# Autodesk Inventor assembly: Head
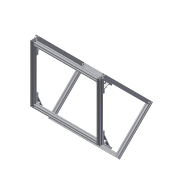
[picture p0: Inventor's stored thumbnail of the model, 180x180]
Saved by Autodesk Inventor 2014 SP1 (Build 180222100, 222)
## iProperties
Created: 2015-02-11
Part Number: Head
Document SubType Name: Assembly
Designer: Simen
Author: Simen
## Documents named in this file (9)
- C:\Users\Simen\Documents\git\Eit\skjellet\Head.iam
- C:\Users\Simen\Documents\git\Eit\skjellet\HBL45TS6hbl45ts6.ipt
- C:\Users\Simen\Documents\git\Eit\skjellet\HBL135TS6.iam
- C:\Users\Simen\Documents\git\Eit\skjellet\KHFS5_2020_386.ipt
- C:\Users\Simen\Documents\git\Eit\skjellet\KHFS5_2020_391.ipt
- C:\Users\Simen\Documents\git\Eit\skjellet\KHFS5_2020_410.ipt
- C:\Users\Simen\Documents\git\Eit\skjellet\HBLFSN5.iam
- C:\Users\Simen\Documents\git\Eit\skjellet\KHFS5_2020_330.ipt
- C:\Users\Simen\Documents\git\Eit\skjellet\KHFS5_2020_101.ipt
## Components (17 placed, 4 different names)
1. HBL45TS6hbl45ts6:1 — Mate:42, Flush:38, Mate:43, Mate:53, Mate:54
2. HBL135TS6:1 [sub-assembly] — Mate:57, Flush:52, Mate:58, Mate:66
3. HBL45TS6hbl45ts6:2 — Mate:41, Flush:39, Mate:44, Mate:55, Mate:56, Flush:51
4. HBL135TS6:2 [sub-assembly] — Mate:69, Flush:67, Mate:72
5. KHFS5-2020-4000:17 — Mate:63, Flush:59, Flush:60, Mate:65, Flush:64, Flush:65
6. KHFS5-2020-4000:18 — Mate:41, Flush:39, Mate:44
7. KHFS5-2020-4000:19 — Mate:42, Flush:38, Mate:43, Flush:50, Flush:56, Mate:62, Flush:58, Flush:61
8. KHFS5-2020-4000:26 — Flush:62, Mate:64, Flush:63, Flush:68, Mate:70, Flush:69
9. KHFS5-2020-4000:27 — Mate:60, Flush:55, Flush:58
10. KHFS5-2020-4000:28 — Mate:59, Flush:53, Flush:54
11. HBLFSN5:1 [sub-assembly] — Mate:61, Flush:57, Mate:68
12. KHFS5-2020-4000:29 — Mate:53, Mate:54, Flush:50, Mate:57, Flush:52, Mate:58, Mate:59, Flush:53, Flush:54, Mate:63, Flush:59, Flush:60
13. KHFS5-2020-4000:30 — Mate:55, Mate:56, Flush:51, Mate:65, Flush:64, Flush:65, Mate:69, Flush:67
14. KHFS5-2020-4000:31 — Mate:60, Flush:55, Flush:56, Mate:61, Flush:57, Mate:62, Flush:61, Flush:62, Mate:64, Flush:63, Mate:67, Flush:66
15. KHFS5-2020-4000:32 — Mate:66, Mate:67, Flush:66, Mate:68
16. KHFS5-2020-4000:33 — Mate:71, Flush:70, Flush:71, Mate:72
17. KHFS5-2020-4000:34 — Flush:68, Mate:70, Flush:69, Mate:71, Flush:70, Flush:71
## Relationships (48: Mate 24, Flush 24)
- Mate:41: HBL45TS6hbl45ts6:2 ↔ KHFS5-2020-4000:18
- Mate:42: HBL45TS6hbl45ts6:1 ↔ KHFS5-2020-4000:19
- Flush:38: HBL45TS6hbl45ts6:1 ↔ KHFS5-2020-4000:19
- Flush:39: HBL45TS6hbl45ts6:2 ↔ KHFS5-2020-4000:18
- Mate:43: HBL45TS6hbl45ts6:1 ↔ KHFS5-2020-4000:19
- Mate:44: HBL45TS6hbl45ts6:2 ↔ KHFS5-2020-4000:18
- Mate:53: HBL45TS6hbl45ts6:1 ↔ KHFS5-2020-4000:29
- Mate:54: HBL45TS6hbl45ts6:1 ↔ KHFS5-2020-4000:29
- Flush:50: KHFS5-2020-4000:19 ↔ KHFS5-2020-4000:29
- Mate:55: HBL45TS6hbl45ts6:2 ↔ KHFS5-2020-4000:30
- Mate:56: HBL45TS6hbl45ts6:2 ↔ KHFS5-2020-4000:30
- Flush:51: HBL45TS6hbl45ts6:2 ↔ KHFS5-2020-4000:30
- Mate:57: HBL135TS6:1 ↔ KHFS5-2020-4000:29
- Flush:52: HBL135TS6:1 ↔ KHFS5-2020-4000:29
- Mate:58: HBL135TS6:1 ↔ KHFS5-2020-4000:29
- Mate:59: KHFS5-2020-4000:28 ↔ KHFS5-2020-4000:29
- Flush:53: KHFS5-2020-4000:28 ↔ KHFS5-2020-4000:29
- Flush:54: KHFS5-2020-4000:28 ↔ KHFS5-2020-4000:29
- Mate:60: KHFS5-2020-4000:27 ↔ KHFS5-2020-4000:31
- Flush:55: KHFS5-2020-4000:27 ↔ KHFS5-2020-4000:31
- Flush:56: KHFS5-2020-4000:19 ↔ KHFS5-2020-4000:31
- Mate:61: HBLFSN5:1 ↔ KHFS5-2020-4000:31
- Flush:57: HBLFSN5:1 ↔ KHFS5-2020-4000:31
- Mate:62: KHFS5-2020-4000:19 ↔ KHFS5-2020-4000:31
- Flush:58: KHFS5-2020-4000:19 ↔ KHFS5-2020-4000:27
- Mate:63: KHFS5-2020-4000:17 ↔ KHFS5-2020-4000:29
- Flush:59: KHFS5-2020-4000:17 ↔ KHFS5-2020-4000:29
- Flush:60: KHFS5-2020-4000:17 ↔ KHFS5-2020-4000:29
- Flush:61: KHFS5-2020-4000:19 ↔ KHFS5-2020-4000:31
- Flush:62: KHFS5-2020-4000:26 ↔ KHFS5-2020-4000:31
- Mate:64: KHFS5-2020-4000:26 ↔ KHFS5-2020-4000:31
- Flush:63: KHFS5-2020-4000:26 ↔ KHFS5-2020-4000:31
- Mate:65: KHFS5-2020-4000:17 ↔ KHFS5-2020-4000:30
- Flush:64: KHFS5-2020-4000:17 ↔ KHFS5-2020-4000:30
- Flush:65: KHFS5-2020-4000:17 ↔ KHFS5-2020-4000:30
- Mate:66: HBL135TS6:1 ↔ KHFS5-2020-4000:32
- Mate:67: KHFS5-2020-4000:31 ↔ KHFS5-2020-4000:32
- Flush:66: KHFS5-2020-4000:31 ↔ KHFS5-2020-4000:32
- Mate:68: HBLFSN5:1 ↔ KHFS5-2020-4000:32
- Mate:69: HBL135TS6:2 ↔ KHFS5-2020-4000:30
- Flush:67: HBL135TS6:2 ↔ KHFS5-2020-4000:30
- Flush:68: KHFS5-2020-4000:26 ↔ KHFS5-2020-4000:34
- Mate:70: KHFS5-2020-4000:26 ↔ KHFS5-2020-4000:34
- Flush:69: KHFS5-2020-4000:26 ↔ KHFS5-2020-4000:34
- Mate:71: KHFS5-2020-4000:33 ↔ KHFS5-2020-4000:34
- Flush:70: KHFS5-2020-4000:33 ↔ KHFS5-2020-4000:34
- Flush:71: KHFS5-2020-4000:33 ↔ KHFS5-2020-4000:34
- Mate:72: HBL135TS6:2 ↔ KHFS5-2020-4000:33
